# Autodesk Inventor assembly: rack_and_pinion
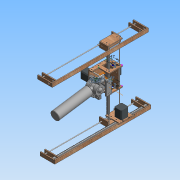
[picture p0: Inventor's stored thumbnail of the model, 180x180]
Saved by Autodesk Inventor 2015 (Build 190159000, 159)
## iProperties
Created: 2014-09-02
Part Number: rack_and_pinion
Document SubType Name: Assembly
Designer: shohei
Author: shohei
## Documents named in this file (19)
- C:\Users\shohei\Documents\Inventor\PlasmaCNCrev3\Workspaces\Workspace\rack_and_pinion.iam
- C:\Users\shohei\Documents\Inventor\PlasmaCNCrev3\Workspaces\Workspace\rack1.ipt
- C:\Users\shohei\Documents\Inventor\PlasmaCNCrev3\Workspaces\Workspace\rack_and_pinion\Design Accelerator\Spur Gears1.iam
- C:\Users\shohei\Documents\Inventor\PlasmaCNCrev3\Workspaces\Workspace\42BYGHM809.ipt
- C:\Users\shohei\Documents\Inventor\PlasmaCNCrev3\Workspaces\Workspace\holder_plate.ipt
- C:\Users\shohei\Documents\Inventor\PlasmaCNCrev3\Workspaces\Workspace\rack_and_pinion_X.iam
- C:\Users\shohei\Documents\Inventor\PlasmaCNCrev3\Workspaces\Workspace\longshaft.ipt
- C:\Users\shohei\Documents\Inventor\PlasmaCNCrev3\Workspaces\Workspace\torchHolder.ipt
- C:\Users\shohei\Documents\Inventor\PlasmaCNCrev3\Workspaces\Workspace\holdersupport.ipt
- C:\Users\shohei\Documents\Inventor\PlasmaCNCrev3\Workspaces\Workspace\main\motor_assembly_z.iam
- C:\Users\shohei\Documents\Inventor\PlasmaCNCrev3\Workspaces\Workspace\holder_sideblock.ipt
- C:\Users\shohei\Documents\Inventor\PlasmaCNCrev3\Workspaces\Workspace\plasmaTorchAssembly.iam
- C:\Users\shohei\Documents\Inventor\PlasmaCNCrev3\Workspaces\Workspace\stopper.ipt
- C:\Users\shohei\Documents\Inventor\PlasmaCNCrev3\Workspaces\Workspace\holder_plate4.ipt
- C:\Users\shohei\Documents\Inventor\PlasmaCNCrev3\slider_box.ipt
- C:\Users\shohei\Documents\Inventor\PlasmaCNCrev3\Workspaces\Workspace\holder_plate_side.ipt
- C:\Users\shohei\Documents\Inventor\PlasmaCNCrev3\Workspaces\Workspace\longshaft2.ipt
- C:\Users\shohei\Documents\Inventor\PlasmaCNCrev3\slider_box2.ipt
- C:\Users\shohei\Documents\Inventor\PlasmaCNCrev3\rail_plate.ipt
## Components (40 placed, 18 different names)
1. rack1:1 — Angle:19, Mate:94, Mate:95, Flush:89, Mate:96, Mate:99, Mate:100
2. Spur Gears:1 [sub-assembly] — Mate:1, Mate:2, Mate:5, Angle:4, Rotational:1
3. 42BYGHM809:1 — Rotational:1, Angle:20, Mate:84, Mate:85
4. rack_and_pinion_X:1 [sub-assembly] — Rotational:8, Angle:22
5. 42BYGHM809:2 — Rotational:8, Angle:12, Mate:12, Mate:13, Mate:14
6. torchHolder:1 — Rotational:14, Insert:1, Angle:14, Insert:2, Angle:15, Insert:3, Angle:16, Insert:4, Angle:17, Angle:18
7. torchHolder:2 — Mate:54, Flush:65, Flush:66
8. holder_plate:3 — Mate:12, Mate:13, Mate:14, Mate:40, Mate:66, Mate:82, Mate:92
9. holdersupport:1 — Mate:40, Mate:46, Flush:54, Rigid:1, Cylindrical:54, Mate:92
10. holdersupport:2 — Mate:67, Flush:70, Flush:78, Flush:79
11. motor_assembly_z:1 [sub-assembly] — Mate:46, Flush:54, Mate:55, Mate:56, Mate:57, Mate:58, Mate:60, Mate:61, Mate:62, Mate:63, Mate:66, Mate:67, Flush:70, Flush:78, Flush:79, Mate:82
12. longshaft:3 — Rigid:1, Rotational:16, Cylindrical:54, Rotational:17
13. holder_sideblock:1 — Insert:1, Angle:14, Mate:59
14. holder_sideblock:2 — Insert:3, Angle:16, Mate:56, Mate:57
15. holder_sideblock:3 — Insert:4, Angle:17
16. holder_sideblock:4 — Mate:54, Flush:65, Flush:66, Insert:2, Angle:15, Mate:55
17. plasmaTorchAssembly:1 [sub-assembly] — Rotational:14
18. stopper:2 — Mate:58, Mate:59, Mate:60
19. stopper:3 — Mate:61, Mate:62, Mate:63
20. holder_plate4:1 — Mate:89, Mate:90, Flush:85
21. holder_plate4:3 — Mate:89, Mate:91, Flush:87, Mate:93, Rotational:17, Rotational:18
22. longshaft:4 — Cylindrical:51, Rotational:18
23. holder_plate4:5 — Cylindrical:51, Rotational:16, Mate:86, Mate:87, Flush:80, Flush:83, Flush:98, Mate:107, Flush:99
24. slider_box:1 — Mate:87, Flush:80, Cylindrical:55, Flush:98
25. holder_plate_side:1 — Angle:21, Mate:84, Mate:85, Angle:22, Mate:86
26. slider_box:2 — Flush:83, Mate:107, Flush:99
27. slider_box:3 — Mate:90, Flush:85, Cylindrical:56, Mate:93
28. slider_box:4 — Mate:91, Flush:87
29. longshaft2:1 — Cylindrical:55, Rotational:19, Rotational:20, Cylindrical:57, Cylindrical:58
30. longshaft2:2 — Cylindrical:56, Rotational:21, Rotational:22
31. slider_box2:1 — Rotational:19, Mate:94, Mate:95, Flush:89, Mate:97, Mate:101, Flush:90, Flush:91
32. slider_box2:2 — Rotational:20, Mate:96, Mate:98, Flush:97
33. slider_box2:3 — Cylindrical:57, Mate:97, Mate:100
34. slider_box2:4 — Cylindrical:58, Mate:98, Mate:99
35. slider_box2:5 — Rotational:21, Angle:23, Mate:102, Flush:92, Flush:93, Flush:94, Mate:104
36. slider_box2:6 — Rotational:22, Angle:24, Mate:105, Flush:95, Flush:96, Flush:97
37. rail_plate:1 — Mate:101, Flush:90, Flush:91
38. rail_plate:2 — Mate:102, Flush:92, Flush:93, Mate:103, Mate:106
39. slider_box2:7 — Mate:103, Flush:94, Mate:104
40. slider_box2:8 — Mate:105, Flush:95, Flush:96, Mate:106
## Relationships (101: Mate 45, Flush 21, Angle 14, RevoluteJoint 10, CylindricalJoint 6, Insert 4, WeldJoint 1)
- Mate:1: Spur Gears:1
- Mate:2: Spur Gears:1
- Mate:5: Spur Gears:1
- Angle:4 (12 deg): Spur Gears:1
- Angle:7 (0 deg)
- Mate:6
- Rotational:1 [RevoluteJoint]: Spur Gears:1 ↔ 42BYGHM809:1
- Rotational:8 [RevoluteJoint]: rack_and_pinion_X:1 ↔ 42BYGHM809:2
- Angle:12 (0 deg): 42BYGHM809:2
- Mate:12: 42BYGHM809:2 ↔ holder_plate:3
- Mate:13: 42BYGHM809:2 ↔ holder_plate:3
- Mate:14: 42BYGHM809:2 ↔ holder_plate:3
- Mate:40: holder_plate:3 ↔ holdersupport:1
- Mate:46: holdersupport:1 ↔ motor_assembly_z:1
- Flush:54: holdersupport:1 ↔ motor_assembly_z:1
- Mate:54: torchHolder:2 ↔ holder_sideblock:4
- Flush:65: torchHolder:2 ↔ holder_sideblock:4
- Flush:66: torchHolder:2 ↔ holder_sideblock:4
- Rotational:14 [RevoluteJoint]: torchHolder:1 ↔ plasmaTorchAssembly:1
- Insert:1: torchHolder:1 ↔ holder_sideblock:1
- Angle:14 (0 deg): torchHolder:1 ↔ holder_sideblock:1
- Insert:2: torchHolder:1 ↔ holder_sideblock:4
- Angle:15 (0 deg): torchHolder:1 ↔ holder_sideblock:4
- Insert:3: torchHolder:1 ↔ holder_sideblock:2
- Angle:16 (0 deg): torchHolder:1 ↔ holder_sideblock:2
- Insert:4: torchHolder:1 ↔ holder_sideblock:3
- Angle:17 (0 deg): torchHolder:1 ↔ holder_sideblock:3
- Angle:18 (0 deg): torchHolder:1
- Mate:55: motor_assembly_z:1 ↔ holder_sideblock:4
- Mate:56: motor_assembly_z:1 ↔ holder_sideblock:2
- Mate:57: motor_assembly_z:1 ↔ holder_sideblock:2
- Mate:58: motor_assembly_z:1 ↔ stopper:2
- Mate:59: holder_sideblock:1 ↔ stopper:2
- Mate:60: motor_assembly_z:1 ↔ stopper:2
- Mate:61: motor_assembly_z:1 ↔ stopper:3
- Mate:62: motor_assembly_z:1 ↔ stopper:3
- Mate:63: motor_assembly_z:1 ↔ stopper:3
- Mate:66: holder_plate:3 ↔ motor_assembly_z:1
- Mate:67: holdersupport:2 ↔ motor_assembly_z:1
- Flush:70: holdersupport:2 ↔ motor_assembly_z:1
- Flush:78: holdersupport:2 ↔ motor_assembly_z:1
- Flush:79: holdersupport:2 ↔ motor_assembly_z:1
- Rigid:1 [WeldJoint]: holdersupport:1 ↔ longshaft:3
- Cylindrical:51: longshaft:4 ↔ holder_plate4:5
- Mate:82: holder_plate:3 ↔ motor_assembly_z:1
- Rotational:16 [RevoluteJoint]: longshaft:3 ↔ holder_plate4:5
- Angle:19 (0 deg): rack1:1
- Angle:20 (0 deg): 42BYGHM809:1
- Angle:21 (0 deg): holder_plate_side:1
- Mate:84: 42BYGHM809:1 ↔ holder_plate_side:1
- Mate:85: 42BYGHM809:1 ↔ holder_plate_side:1
- Angle:22 (180 deg): rack_and_pinion_X:1 ↔ holder_plate_side:1
- Mate:86 (20 mm): holder_plate4:5 ↔ holder_plate_side:1
- Mate:87: holder_plate4:5 ↔ slider_box:1
- Flush:80: holder_plate4:5 ↔ slider_box:1
- Flush:83: holder_plate4:5 ↔ slider_box:2
- Mate:89 (20 mm): holder_plate4:1 ↔ holder_plate4:3
- Mate:90: holder_plate4:1 ↔ slider_box:3
- Flush:85: holder_plate4:1 ↔ slider_box:3
- Mate:91: holder_plate4:3 ↔ slider_box:4
- Flush:87: holder_plate4:3 ↔ slider_box:4
- Cylindrical:54: holdersupport:1 ↔ longshaft:3
- Mate:92: holder_plate:3 ↔ holdersupport:1
- Cylindrical:55: slider_box:1 ↔ longshaft2:1
- Cylindrical:56: slider_box:3 ↔ longshaft2:2
- Mate:93: holder_plate4:3 ↔ slider_box:3
- Rotational:17 [RevoluteJoint]: longshaft:3 ↔ holder_plate4:3
- Rotational:18 [RevoluteJoint]: holder_plate4:3 ↔ longshaft:4
- Rotational:19 [RevoluteJoint]: longshaft2:1 ↔ slider_box2:1
- Mate:94: rack1:1 ↔ slider_box2:1
- Mate:95: rack1:1 ↔ slider_box2:1
- Flush:89: rack1:1 ↔ slider_box2:1
- Rotational:20 [RevoluteJoint]: longshaft2:1 ↔ slider_box2:2
- Mate:96: rack1:1 ↔ slider_box2:2
- Cylindrical:57: longshaft2:1 ↔ slider_box2:3
- Mate:97 (20 mm): slider_box2:1 ↔ slider_box2:3
- Cylindrical:58: longshaft2:1 ↔ slider_box2:4
- Mate:98 (20 mm): slider_box2:2 ↔ slider_box2:4
- Mate:99: rack1:1 ↔ slider_box2:4
- Mate:100: rack1:1 ↔ slider_box2:3
- Mate:101: slider_box2:1 ↔ rail_plate:1
- Flush:90: slider_box2:1 ↔ rail_plate:1
- Flush:91: slider_box2:1 ↔ rail_plate:1
- Rotational:21 [RevoluteJoint]: longshaft2:2 ↔ slider_box2:5
- Rotational:22 [RevoluteJoint]: longshaft2:2 ↔ slider_box2:6
- Angle:23 (0 deg): slider_box2:5
- Angle:24 (0 deg): slider_box2:6
- Mate:102: slider_box2:5 ↔ rail_plate:2
- Flush:92: slider_box2:5 ↔ rail_plate:2
- Flush:93: slider_box2:5 ↔ rail_plate:2
- Mate:103: rail_plate:2 ↔ slider_box2:7
- Flush:94: slider_box2:5 ↔ slider_box2:7
- Mate:104 (20 mm): slider_box2:5 ↔ slider_box2:7
- Mate:105 (20 mm): slider_box2:6 ↔ slider_box2:8
- Flush:95: slider_box2:6 ↔ slider_box2:8
- Flush:96: slider_box2:6 ↔ slider_box2:8
- Mate:106: rail_plate:2 ↔ slider_box2:8
- Flush:97: slider_box2:2 ↔ slider_box2:6
- Flush:98: holder_plate4:5 ↔ slider_box:1
- Mate:107: holder_plate4:5 ↔ slider_box:2
- Flush:99: holder_plate4:5 ↔ slider_box:2
